# Autodesk Inventor assembly: Assembly1
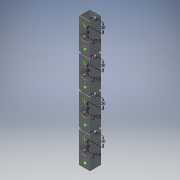
[picture p0: Inventor's stored thumbnail of the model, 180x180]
Saved by Autodesk Inventor 2018 (Build 220112000, 112)
## iProperties
Created: 2017-09-14
Part Number: Assembly1
Material: 一般
Document SubType Name: Assembly
Designer: Kenta
Author: Kenta
## Documents named in this file (2)
- C:\Users\Kenta\Documents\workspace\rbbr\cart\前足改\Assembly1.iam
- C:\Users\Kenta\Documents\workspace\rbbr\cart\前足改\軸受上用.ipt
## Components (8 placed, 1 different names)
1. 軸受上用:1 — リジッド:1
2. 軸受上用:2 — リジッド:1, リジッド:3
3. 軸受上用:3 — リジッド:3
4. 軸受上用:4 — リジッド:7
5. 軸受上用:5 — リジッド:7
6. 軸受上用:6 — リジッド:6
7. 軸受上用:7 — リジッド:6
8. 軸受上用:8
## Relationships (7: WeldJoint 7)
- リジッド:1 [WeldJoint]: 軸受上用:1 ↔ 軸受上用:2
- [WeldJoint]: 軸受上用:3 ↔ 軸受上用:4
- リジッド:3 [WeldJoint] (5 mm): 軸受上用:2 ↔ 軸受上用:3
- [WeldJoint]: 軸受上用:5 ↔ 軸受上用:6
- [WeldJoint]: 軸受上用:7 ↔ 軸受上用:8
- リジッド:6 [WeldJoint] (5 mm): 軸受上用:6 ↔ 軸受上用:7
- リジッド:7 [WeldJoint] (5 mm): 軸受上用:4 ↔ 軸受上用:5
## Named parameters: d9_d8 = 0 mm, d11_d8 = 0 mm, d12_d9_d8 = 0 mm, d13_d10 = 5 mm
